# Autodesk Inventor assembly: FRC210-1S
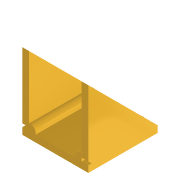
[picture p0: Inventor's stored thumbnail of the model, 180x180]
Saved by Autodesk Inventor 2020 (Build 240168000, 168)
## iProperties
Created: 2020-02-19
Part Number: FRC210-1S
Document SubType Name: Weldment
Designer: Juan Carlos Botero
Mass: 65.461 g
Surface Area: 210.033 cm^2
Volume: 48.0913 cm^3
Density: 1.36118 g/cm^3
Weld Material: Aluminum 6061, Welded
Author: Juan Carlos Botero
Title: SOPORTE FIJO
## Documents named in this file (3)
- D:\Drives\OneDrive\Carlos_2\02 TRABAJOS\MULTIPLO\Conveyor\ENSAMBLE - Copy\Tensor.iam
- D:\Drives\OneDrive\Carlos_2\02 TRABAJOS\MULTIPLO\Conveyor\ENSAMBLE - Copy\Placa central soporte.ipt
- D:\Drives\OneDrive\Carlos_2\02 TRABAJOS\MULTIPLO\Conveyor\ENSAMBLE - Copy\Refuerzo soporte.ipt
## Components (3 placed, 2 different names)
1. Placa central soporte:1 — Mate:2, Flush:3, Flush:4, Mate:5, Flush:6, Flush:7, Flush:8, Flush:9
2. Refuerzo soporte:1 — Mate:2, Flush:3, Flush:4, Flush:5
3. Refuerzo soporte:2 — Mate:5, Flush:5, Flush:6
## Relationships (9: Flush 7, Mate 2)
- Mate:2: Placa central soporte:1 ↔ Refuerzo soporte:1
- Flush:3: Placa central soporte:1 ↔ Refuerzo soporte:1
- Flush:4: Placa central soporte:1 ↔ Refuerzo soporte:1
- Mate:5: Placa central soporte:1 ↔ Refuerzo soporte:2
- Flush:5: Refuerzo soporte:1 ↔ Refuerzo soporte:2
- Flush:6: Placa central soporte:1 ↔ Refuerzo soporte:2
- Flush:7: Placa central soporte:1
- Flush:8: Placa central soporte:1
- Flush:9: Placa central soporte:1
